# Autodesk Inventor assembly: placering af top vange-endeplade på stillads
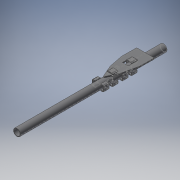
[picture p0: Inventor's stored thumbnail of the model, 180x180]
Saved by Autodesk Inventor 2018 (Build 220112000, 112)
## iProperties
Created: 2019-10-12
Part Number: placering af top vange-endeplade på stillads
Document SubType Name: Assembly
Designer: loppen
Author: loppen
## Documents named in this file (3)
- Z:\trappe\placering af top vange-endeplade på stillads.iam
- Z:\trappe\søjle\stilladssøjle.iam
- Z:\trappe\top vange-endeplade.ipt
## Components (2 placed, 2 different names)
1. stilladssøjle:1 [sub-assembly] — Mate:1, Mate:2
2. top vange-endeplade:1 — Mate:1, Mate:2
## Relationships (2: Mate 2)
- Mate:1: stilladssøjle:1 ↔ top vange-endeplade:1
- Mate:2: stilladssøjle:1 ↔ top vange-endeplade:1
